# Autodesk Inventor assembly: Switching power supply
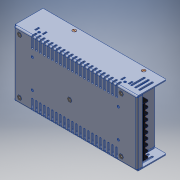
[picture p0: Inventor's stored thumbnail of the model, 180x180]
Saved by Autodesk Inventor 2016 (Build 200138000, 138)
## iProperties
Created: 2013-12-07
Part Number: Switching power supply
Description: STEP AP214
Document SubType Name: Assembly
Designer: Mathias L. Kjeldgaard
Sending System: SolidWorks 2012
Preprocessor: SwSTEP 2.0
Title: Switching power supply.STEP
Author: John van der Sanden
Revision Number: ANY
## Documents named in this file (13)
- C:\Users\PowerStation9000\AppData\Local\Autodesk\Autodesk Sync\Cloud\mathiaslk\UltiBot mk2 rev2\Importerede komponenter\PSU\Switching power supply.iam
- C:\Users\PowerStation9000\AppData\Local\Autodesk\Autodesk Sync\Cloud\mathiaslk\UltiBot mk2 rev2\Importerede komponenter\PSU\SWP (Basis).ipt
- C:\Users\PowerStation9000\AppData\Local\Autodesk\Autodesk Sync\Cloud\mathiaslk\UltiBot mk2 rev2\Importerede komponenter\PSU\SWP (Deksel).ipt
- C:\Users\PowerStation9000\AppData\Local\Autodesk\Autodesk Sync\Cloud\mathiaslk\UltiBot mk2 rev2\Importerede komponenter\PSU\Slotted Countersunk Flat Head Screw_DIN_ISO 2009 - M3 x 5 --- 5N.ipt
- C:\Users\PowerStation9000\AppData\Local\Autodesk\Autodesk Sync\Cloud\mathiaslk\UltiBot mk2 rev2\Importerede komponenter\PSU\Body 60mm fan.ipt
- C:\Users\PowerStation9000\AppData\Local\Autodesk\Autodesk Sync\Cloud\mathiaslk\UltiBot mk2 rev2\Importerede komponenter\PSU\Propellor 60mm fan.ipt
- C:\Users\PowerStation9000\AppData\Local\Autodesk\Autodesk Sync\Cloud\mathiaslk\UltiBot mk2 rev2\Importerede komponenter\PSU\Slotted Countersunk Flat Head Screw_DIN_ISO 2009 - M3 x 20 --- 20N.ipt
- C:\Users\PowerStation9000\AppData\Local\Autodesk\Autodesk Sync\Cloud\mathiaslk\UltiBot mk2 rev2\Importerede komponenter\PSU\SWP (M3 moer).ipt
- C:\Users\PowerStation9000\AppData\Local\Autodesk\Autodesk Sync\Cloud\mathiaslk\UltiBot mk2 rev2\Importerede komponenter\PSU\SWP (PCB).ipt
- C:\Users\PowerStation9000\AppData\Local\Autodesk\Autodesk Sync\Cloud\mathiaslk\UltiBot mk2 rev2\Importerede komponenter\PSU\SWP (Montage draad).ipt
- C:\Users\PowerStation9000\AppData\Local\Autodesk\Autodesk Sync\Cloud\mathiaslk\UltiBot mk2 rev2\Importerede komponenter\PSU\SWP (Montage draad 2).ipt
- C:\Users\PowerStation9000\AppData\Local\Autodesk\Autodesk Sync\Cloud\mathiaslk\UltiBot mk2 rev2\Importerede komponenter\PSU\Slotted Cheese Head Screw_DIN_ISO 1207 - M4 x 5 --- 5N.ipt
- C:\Users\PowerStation9000\AppData\Local\Autodesk\Autodesk Sync\Cloud\mathiaslk\UltiBot mk2 rev2\Importerede komponenter\PSU\SWP (switch).ipt
## Components (46 placed, 25 different names)
1. SWP (Basis)_1 — Insert:2, Insert:3, Insert:4, Insert:5, Insert:6, Insert:7, Mate:4, Flush:2, Mate:5, Mate:6, Mate:7, Flush:3, Mate:12, Mate:13, Mate:14
2. SWP (Deksel)_2 — Mate:3, Flush:1, Insert:1, Mate:17, Mate:18, Mate:19, Mate:20
3. Slotted Countersunk Flat Head Screw_DIN_ISO 2009 - M3 x 5 --- 5N_3 — Insert:7
4. Slotted Countersunk Flat Head Screw_DIN_ISO 2009 - M3 x 5 --- 5N_4 — Insert:6
5. Slotted Countersunk Flat Head Screw_DIN_ISO 2009 - M3 x 5 --- 5N_5 — Insert:3, Mate:19
6. Slotted Countersunk Flat Head Screw_DIN_ISO 2009 - M3 x 5 --- 5N_6 — Insert:2, Mate:18
7. Slotted Countersunk Flat Head Screw_DIN_ISO 2009 - M3 x 5 --- 5N_7 — Insert:5
8. Slotted Countersunk Flat Head Screw_DIN_ISO 2009 - M3 x 5 --- 5N_8 — Insert:4, Mate:20
9. Body 60mm fan_9 — Mate:1, Mate:2, Mate:15, Mate:16, Mate:17
10. Propellor 60mm fan_10 — Mate:1, Mate:2
11. Slotted Countersunk Flat Head Screw_DIN_ISO 2009 - M3 x 20 --- 20N_11 — Mate:3, Flush:1, Mate:15
12. Slotted Countersunk Flat Head Screw_DIN_ISO 2009 - M3 x 20 --- 20N_12 — Insert:1, Mate:16
13. SWP (M3 moer)_13
14. SWP (M3 moer)_14
15. SWP (M3 moer)_15
16. SWP (M3 moer)_16
17. SWP (M3 moer)_17
18. SWP (PCB)_18 — Mate:4, Flush:2, Mate:5, Mate:6, Mate:7, Flush:3, Mate:9, Mate:10, Mate:11
19. SWP (switch)_46 — Mate:12, Mate:13, Mate:14
20. SWP (Montage draad)_29 — Flush:4, Flush:5, Mate:8, Mate:10, Mate:11
21. SWP (Montage draad 2)_37 — Flush:4, Flush:5, Mate:8, Insert:8
22. Slotted Cheese Head Screw_DIN_ISO 1207 - M4 x 5 --- 5N_45 — Insert:8, Mate:9
23. SWP (Montage draad):10
24. SWP (Montage draad 2):10
25. Slotted Cheese Head Screw_DIN_ISO 1207 - M4 x 5 --- 5N:10
26. SWP (Montage draad):11
27. SWP (Montage draad 2):11
28. Slotted Cheese Head Screw_DIN_ISO 1207 - M4 x 5 --- 5N:11
29. SWP (Montage draad):12
30. SWP (Montage draad 2):12
31. Slotted Cheese Head Screw_DIN_ISO 1207 - M4 x 5 --- 5N:12
32. SWP (Montage draad):13
33. SWP (Montage draad 2):13
34. Slotted Cheese Head Screw_DIN_ISO 1207 - M4 x 5 --- 5N:13
35. SWP (Montage draad):14
36. SWP (Montage draad 2):14
37. Slotted Cheese Head Screw_DIN_ISO 1207 - M4 x 5 --- 5N:14
38. SWP (Montage draad):15
39. SWP (Montage draad 2):15
40. Slotted Cheese Head Screw_DIN_ISO 1207 - M4 x 5 --- 5N:15
41. SWP (Montage draad):16
42. SWP (Montage draad 2):16
43. Slotted Cheese Head Screw_DIN_ISO 1207 - M4 x 5 --- 5N:16
44. SWP (Montage draad):17
45. SWP (Montage draad 2):17
46. Slotted Cheese Head Screw_DIN_ISO 1207 - M4 x 5 --- 5N:17
## Component patterns: (9 elements, first: SWP (Montage draad)_29 + SWP (Montage draad 2)_37 + Slotted Cheese Head Screw_DIN_ISO 1207 - M4 x 5 --- 5N_45)
## Relationships (33: Mate 20, Insert 8, Flush 5)
- Mate:1: Body 60mm fan_9 ↔ Propellor 60mm fan_10
- Mate:2: Body 60mm fan_9 ↔ Propellor 60mm fan_10
- Mate:3: SWP (Deksel)_2 ↔ Slotted Countersunk Flat Head Screw_DIN_ISO 2009 - M3 x 20 --- 20N_11
- Flush:1: SWP (Deksel)_2 ↔ Slotted Countersunk Flat Head Screw_DIN_ISO 2009 - M3 x 20 --- 20N_11
- Insert:1: SWP (Deksel)_2 ↔ Slotted Countersunk Flat Head Screw_DIN_ISO 2009 - M3 x 20 --- 20N_12
- Insert:2: SWP (Basis)_1 ↔ Slotted Countersunk Flat Head Screw_DIN_ISO 2009 - M3 x 5 --- 5N_6
- Insert:3: SWP (Basis)_1 ↔ Slotted Countersunk Flat Head Screw_DIN_ISO 2009 - M3 x 5 --- 5N_5
- Insert:4: SWP (Basis)_1 ↔ Slotted Countersunk Flat Head Screw_DIN_ISO 2009 - M3 x 5 --- 5N_8
- Insert:5: SWP (Basis)_1 ↔ Slotted Countersunk Flat Head Screw_DIN_ISO 2009 - M3 x 5 --- 5N_7
- Insert:6: SWP (Basis)_1 ↔ Slotted Countersunk Flat Head Screw_DIN_ISO 2009 - M3 x 5 --- 5N_4
- Insert:7: SWP (Basis)_1 ↔ Slotted Countersunk Flat Head Screw_DIN_ISO 2009 - M3 x 5 --- 5N_3
- Mate:4 (-9.75 mm): SWP (Basis)_1 ↔ SWP (PCB)_18
- Flush:2 (1.75 mm): SWP (Basis)_1 ↔ SWP (PCB)_18
- Mate:5: SWP (Basis)_1 ↔ SWP (PCB)_18
- Mate:6 (6.156 mm): SWP (Basis)_1 ↔ SWP (PCB)_18
- Mate:7 (17.8 mm): SWP (Basis)_1 ↔ SWP (PCB)_18
- Flush:3 (3.25 mm): SWP (Basis)_1 ↔ SWP (PCB)_18
- Flush:4: SWP (Montage draad)_29 ↔ SWP (Montage draad 2)_37
- Flush:5: SWP (Montage draad)_29 ↔ SWP (Montage draad 2)_37
- Mate:8: SWP (Montage draad)_29 ↔ SWP (Montage draad 2)_37
- Insert:8: SWP (Montage draad 2)_37 ↔ Slotted Cheese Head Screw_DIN_ISO 1207 - M4 x 5 --- 5N_45
- Mate:9: SWP (PCB)_18 ↔ Slotted Cheese Head Screw_DIN_ISO 1207 - M4 x 5 --- 5N_45
- Mate:10: SWP (PCB)_18 ↔ SWP (Montage draad)_29
- Mate:11: SWP (PCB)_18 ↔ SWP (Montage draad)_29
- Mate:12: SWP (Basis)_1 ↔ SWP (switch)_46
- Mate:13: SWP (Basis)_1 ↔ SWP (switch)_46
- Mate:14: SWP (Basis)_1 ↔ SWP (switch)_46
- Mate:15: Body 60mm fan_9 ↔ Slotted Countersunk Flat Head Screw_DIN_ISO 2009 - M3 x 20 --- 20N_11
- Mate:16: Body 60mm fan_9 ↔ Slotted Countersunk Flat Head Screw_DIN_ISO 2009 - M3 x 20 --- 20N_12
- Mate:17: SWP (Deksel)_2 ↔ Body 60mm fan_9
- Mate:18: SWP (Deksel)_2 ↔ Slotted Countersunk Flat Head Screw_DIN_ISO 2009 - M3 x 5 --- 5N_6
- Mate:19: SWP (Deksel)_2 ↔ Slotted Countersunk Flat Head Screw_DIN_ISO 2009 - M3 x 5 --- 5N_5
- Mate:20: SWP (Deksel)_2 ↔ Slotted Countersunk Flat Head Screw_DIN_ISO 2009 - M3 x 5 --- 5N_8
